# Autodesk Inventor assembly: fff
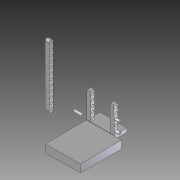
[picture p0: Inventor's stored thumbnail of the model, 180x180]
Saved by Autodesk Inventor 2015 (Build 190159000, 159)
## iProperties
Created: 2015-01-15
Part Number: fff
Document SubType Name: Assembly
Designer: Tucker
Author: Tucker
## Documents named in this file (6)
- C:\Users\Tucker\Documents\GitHub\frc2015\CAD\fff.iam
- C:\Users\Tucker\Documents\GitHub\frc2015\CAD\chasse.ipt
- C:\Users\Tucker\Documents\GitHub\frc2015\CAD\pole.ipt
- C:\Users\Tucker\Documents\GitHub\frc2015\CAD\box_forklift.ipt
- C:\Users\Tucker\Documents\GitHub\frc2015\CAD\axle_word_used_loosely.ipt
- C:\Users\Tucker\Documents\GitHub\frc2015\CAD\gripper_mc_dipper.ipt
## Components (8 placed, 5 different names)
1. chasse:1 — Mate:2, Flush:3, Flush:4
2. pole:2 — Mate:2, Flush:3, Flush:4
3. box_forklift:1 — Mate:13, Flush:8, Flush:9, Mate:14, Flush:10, Flush:11
4. axle_word_used_loosely:2
5. gripper_mc_dipper:1 — Mate:13, Flush:8, Flush:9, Mate:19, Mate:20
6. gripper_mc_dipper:2 — Mate:14, Flush:10, Flush:11
7. axle_word_used_loosely:5 — Mate:20
8. axle_word_used_loosely:6 — Mate:19
## Relationships (11: Flush 6, Mate 5)
- Mate:2: chasse:1 ↔ pole:2
- Flush:3: chasse:1 ↔ pole:2
- Flush:4: chasse:1 ↔ pole:2
- Mate:13: box_forklift:1 ↔ gripper_mc_dipper:1
- Flush:8: box_forklift:1 ↔ gripper_mc_dipper:1
- Flush:9: box_forklift:1 ↔ gripper_mc_dipper:1
- Mate:14: box_forklift:1 ↔ gripper_mc_dipper:2
- Flush:10: box_forklift:1 ↔ gripper_mc_dipper:2
- Flush:11: box_forklift:1 ↔ gripper_mc_dipper:2
- Mate:19: gripper_mc_dipper:1 ↔ axle_word_used_loosely:6
- Mate:20: gripper_mc_dipper:1 ↔ axle_word_used_loosely:5
